# Autodesk Inventor assembly: FMS90mm12Blade8SAssly v7
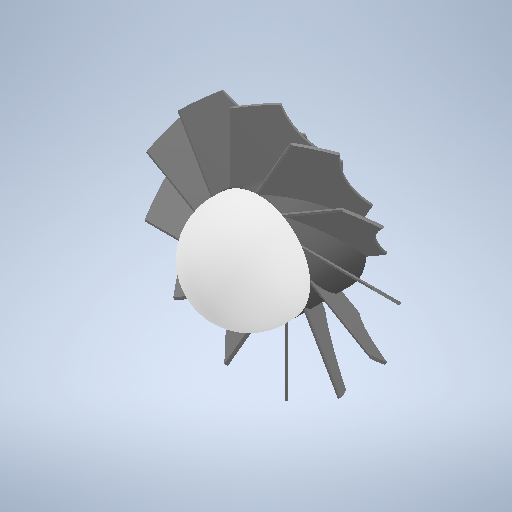
[picture p0: Inventor's stored thumbnail of the model, 512x512]
Saved by Autodesk Inventor 2026.2 (Build 302298010, 298A)
## iProperties
Created: 2022-11-03
Part Number: FMS90mm12Blade8SAssly v7
Document SubType Name: Assembly
Designer: tngzj
Sending System: Autodesk Translation Framework v11.17.0.187
Preprocessor: ST-DEVELOPER v19.2
Title: FMS90mm12Blade8SAssly v7.step
## Documents named in this file (3)
- C:\Transformer-rl-retro-propulsion\CAD\v1\References\FMS90mm12Blade8SAssly v7\FMS90mm12Blade8SAssly v7\FMS90mm12Blade8SAssly v7.iam
- C:\Transformer-rl-retro-propulsion\CAD\v1\References\FMS90mm12Blade8SAssly v7\FMS90mm12Blade8SAssly v7\FMS90mm12BladeFan v3.iam
- C:\Transformer-rl-retro-propulsion\CAD\v1\References\FMS90mm12Blade8SAssly v7\FMS90mm12Blade8SAssly v7\FMS90mm12Blade8SSpinner v4.iam
## Components (2 placed, 2 different names)
1. FMS90mm12BladeFan v3:1 [sub-assembly] — Mate:3, Mate:4
2. FMS90mm12Blade8SSpinner v4:1 [sub-assembly] — Mate:3, Mate:4
## Relationships (2: Mate 2)
- Mate:3: FMS90mm12BladeFan v3:1 ↔ FMS90mm12Blade8SSpinner v4:1
- Mate:4: FMS90mm12BladeFan v3:1 ↔ FMS90mm12Blade8SSpinner v4:1
